# Autodesk Inventor assembly: armrest
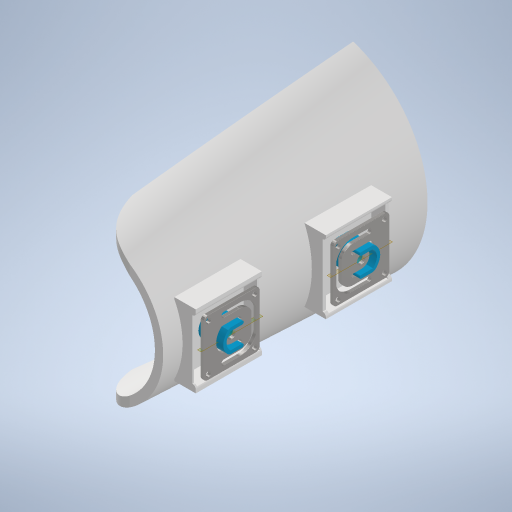
[picture p0: Inventor's stored thumbnail of the model, 512x512]
Saved by Autodesk Inventor 2024 (Build 280153000, 153)
## iProperties
Created: 2023-09-04
Part Number: armrest
Document SubType Name: Assembly
Designer: Pintu
Author: Pintu
## Documents named in this file (4)
- D:\CMC\my_inventor\ArmBo_v2\armrest.iam
- D:\CMC\my_inventor\ArmBo_v2\load_cell_holder.ipt
- D:\CMC\my_inventor\ArmBo_v2\cuff.ipt
- D:\CMC\my_inventor\ArmBo_v2\spuare_load_cell.ipt
## Components (5 placed, 3 different names)
1. cuff:1 — Mate:1, Mate:5
2. spuare_load_cell:1 — Mate:2
3. load_cell_holder:1 — Mate:1, Mate:2
4. load_cell_holder:2 — Mate:5, Mate:6
5. spuare_load_cell:2 — Mate:6
## Relationships (4: Mate 4)
- Mate:1: cuff:1 ↔ load_cell_holder:1
- Mate:2: spuare_load_cell:1 ↔ load_cell_holder:1
- Mate:5: cuff:1 ↔ load_cell_holder:2
- Mate:6: load_cell_holder:2 ↔ spuare_load_cell:2
